# Autodesk Inventor assembly: Ensemble_main
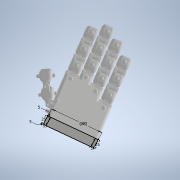
[picture p0: Inventor's stored thumbnail of the model, 180x180]
Saved by Autodesk Inventor 2022 (Build 260153000, 153)
## iProperties
Created: 2022-03-12
Part Number: Ensemble_main
Document SubType Name: Assembly
Designer: timot
Author: timot
## Documents named in this file (5)
- D:\Timothee\Cours\ESEO\P2\TIPE\3D\Main TIPE\Ensemble_main.iam
- D:\Timothee\Cours\ESEO\P2\TIPE\3D\Main TIPE\Phalange.ipt
- Phalange.ipt
- D:\Timothee\Cours\ESEO\P2\TIPE\3D\Main TIPE\Phalange - Bout.ipt
- D:\Timothee\Cours\ESEO\P2\TIPE\3D\Main TIPE\Main-v2.ipt
## Components (15 placed, 2 different names)
1. Phalange:1 — Rotation:2, Rotation:28
2. Phalange:2 — Rotation:2, Rotation:19
3. Phalange:3 — Rotation:18, Rotation:27
4. Phalange:6 — Rotation:6, Rotation:26
5. Phalange:7 — Rotation:6, Rotation:21
6. Phalange:12 — Rotation:10, Rotation:25
7. Phalange:13 — Rotation:10, Rotation:22
8. Phalange:15 — Rotation:15, Rotation:24
9. Phalange:16 — Rotation:15, Rotation:20
10. Phalange:17 — Rotation:18
11. Phalange:18 — Rotation:19
12. Phalange:19 — Rotation:20
13. Phalange:20 — Rotation:21
14. Phalange:21 — Rotation:22
15. Main-v2:1 — Rotation:24, Rotation:26, Rotation:25, Rotation:27, Rotation:28
## Relationships (14: RevoluteJoint 14)
- Rotation:2 [RevoluteJoint] (-0.3 mm): Phalange:1 ↔ Phalange:2
- Rotation:6 [RevoluteJoint] (-0.3 mm): Phalange:6 ↔ Phalange:7
- Rotation:10 [RevoluteJoint] (-0.3 mm): Phalange:12 ↔ Phalange:13
- Rotation:15 [RevoluteJoint] (-0.3 mm): Phalange:15 ↔ Phalange:16
- Rotation:18 [RevoluteJoint] (-0.3 mm): Phalange:3 ↔ Phalange:17
- Rotation:19 [RevoluteJoint] (-0.3 mm): Phalange:2 ↔ Phalange:18
- Rotation:20 [RevoluteJoint] (-0.3 mm): Phalange:16 ↔ Phalange:19
- Rotation:21 [RevoluteJoint] (-0.3 mm): Phalange:7 ↔ Phalange:20
- Rotation:22 [RevoluteJoint] (-0.3 mm): Phalange:13 ↔ Phalange:21
- Rotation:24 [RevoluteJoint] (-0.3 mm): Phalange:15 ↔ Main-v2:1
- Rotation:26 [RevoluteJoint] (-0.3 mm): Phalange:6 ↔ Main-v2:1
- Rotation:25 [RevoluteJoint] (-0.3 mm): Phalange:12 ↔ Main-v2:1
- Rotation:27 [RevoluteJoint] (-0.3 mm): Phalange:3 ↔ Main-v2:1
- Rotation:28 [RevoluteJoint] (-0.3 mm): Phalange:1 ↔ Main-v2:1
## Named parameters: d70_d52 = -0.3 mm, d71_d53 = -0.322935 deg, d72_d54 = 0 deg, d73_d55 = -83 deg, d86_d52 = -0.3 mm, d87_d53 = -0.323081 deg, d88_d54 = 0 deg, d89_d55 = -83 deg, d120_d52 = -0.3 mm, d121_d53 = -0.505856 deg, d122_d54 = 0 deg, d123_d55 = -83 deg
